# Autodesk Inventor assembly: ASY PRS 1200-54 FDS way3_1600
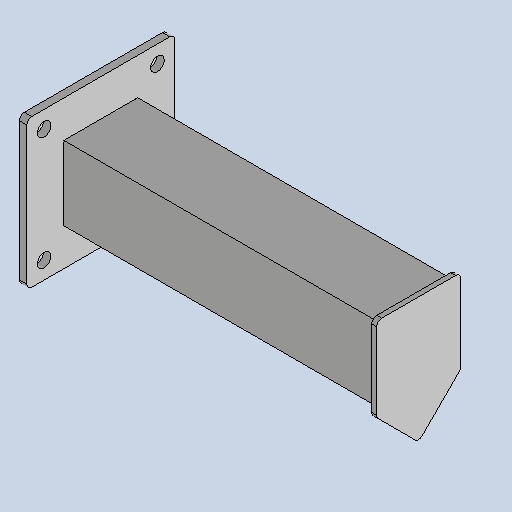
[picture p0: Inventor's stored thumbnail of the model, 512x512]
Saved by Autodesk Inventor 2025.3 (Build 293356030, 356C)
## iProperties
Created: 2025-07-02
Part Number: ASY PRS 1200-54 FDS way3_1600
Document SubType Name: Assembly
Designer: admin
Author: user
## Documents named in this file (4)
- C:\Users\pokla\Documents\Inventor\PRS-Purovskii\Model\PRS-filter 1200\ASY PRS 1200-54 FDS way3_1600.iam
- C:\Users\pokla\Documents\Inventor\PRS-Purovskii\Model\PRS-filter 1200\PRS 1200-54-01 FDS 1200 way tube 3.ipt
- C:\Users\pokla\Documents\Inventor\PRS-Purovskii\Model\PRS-filter 1200\PRS 1200-52-03 FDS 1000 CUP 1.ipt
- C:\Users\pokla\Documents\Inventor\PRS-Purovskii\Model\PRS-filter 1200\PRS 1200-52-04 FDS Way FLANGE.ipt
## Components (3 placed, 3 different names)
1. PNS 1663 FDS 1200 way tube 3.ipt:1 — Rigid:7, Rigid:8
2. PNS 1666 FDS 1000 CUP 1.ipt:1 — Rigid:7
3. SLM 1425 FDS Way FLANGE:1 — Rigid:8
## Relationships (2: WeldJoint 2)
- Rigid:7 [WeldJoint]: PNS 1663 FDS 1200 way tube 3.ipt:1 ↔ PNS 1666 FDS 1000 CUP 1.ipt:1
- Rigid:8 [WeldJoint]: PNS 1663 FDS 1200 way tube 3.ipt:1 ↔ SLM 1425 FDS Way FLANGE:1
